# Autodesk Inventor assembly: SliddingAssembly
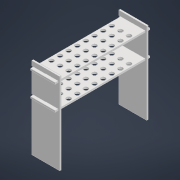
[picture p0: Inventor's stored thumbnail of the model, 180x180]
Saved by Autodesk Inventor 2021.3 (Build 253353000, 353)
## iProperties
Created: 2019-08-12
Part Number: SliddingAssembly
Document SubType Name: Assembly
Designer: eugen
Author: eugen
## Documents named in this file (3)
- C:\Users\eugen\GitHub\ChromatographyRacks\FinalAssembly.iam
- C:\Users\eugen\GitHub\ChromatographyRacks\Rack.ipt
- C:\Users\eugen\GitHub\ChromatographyRacks\Sides.ipt
## Components (4 placed, 2 different names)
1. Rack:1 — Mate:15, Mate:16, Mate:17
2. Sides:1
3. Rack:2 — Mate:18, Mate:19, Mate:20
4. Sides:2 — Mate:15, Mate:16, Mate:17, Mate:18, Mate:19, Mate:20
## Relationships (6: Mate 6)
- Mate:15: Rack:1 ↔ Sides:2
- Mate:16: Rack:1 ↔ Sides:2
- Mate:17: Rack:1 ↔ Sides:2
- Mate:18: Rack:2 ↔ Sides:2
- Mate:19: Rack:2 ↔ Sides:2
- Mate:20: Rack:2 ↔ Sides:2
